# Autodesk Inventor assembly: Ensamble_AX12
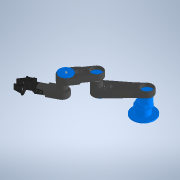
[picture p0: Inventor's stored thumbnail of the model, 180x180]
Saved by Autodesk Inventor 2021 (Build 250183000, 183)
## iProperties
Created: 2022-06-07
Part Number: Ensamble_AX12
Document SubType Name: Assembly
Designer: Alcatraz
Author: Alcatraz
## Documents named in this file (5)
- F:\Tesis\TESIS\Lista_\Ensamble_AX12.iam
- F:\Tesis\TESIS\Lista_\Eslabon_1.iam
- F:\Tesis\TESIS\Lista_\Eslabon_2.iam
- F:\Tesis\TESIS\Lista_\Eslabon_3.iam
- F:\Tesis\TESIS\Lista_\Base\Base_AX12.iam
## Components (4 placed, 4 different names)
1. Eslabon_1:1 [sub-assembly] — De rotación:1, De rotación:2
2. Eslabon_2:1 [sub-assembly] — De rotación:2, De rotación:3
3. Eslabon_3:1 [sub-assembly] — De rotación:3
4. Base_AX12:1 [sub-assembly] — De rotación:1
## Relationships (3: RevoluteJoint 3)
- De rotación:1 [RevoluteJoint]: Eslabon_1:1 ↔ Base_AX12:1
- De rotación:2 [RevoluteJoint]: Eslabon_1:1 ↔ Eslabon_2:1
- De rotación:3 [RevoluteJoint]: Eslabon_2:1 ↔ Eslabon_3:1
